# Autodesk Inventor assembly: enc-BackPanel Unten HF-Durchlass - Assembly
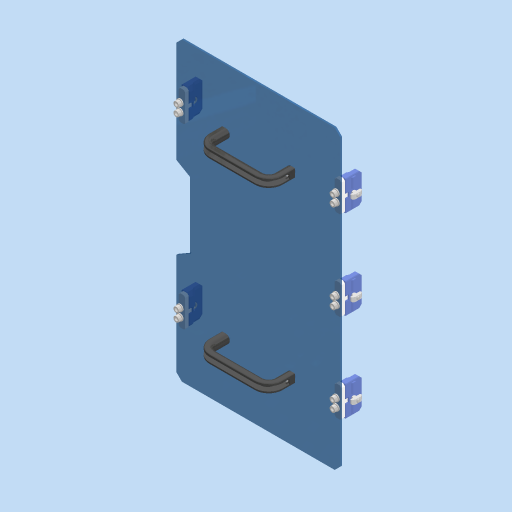
[picture p0: Inventor's stored thumbnail of the model, 512x512]
Saved by Autodesk Inventor 2023.2 (Build 272271000, 271)
## iProperties
Created: 2023-12-04
Part Number: enc-BackPanel Unten HF-Durchlass - Assembly
Document SubType Name: Assembly
Designer: Nils Bade
Author: Nils Bade
## Documents named in this file (4)
- C:\Users\nilsb\Documents\Inventor\Projektarbeit-Bade\Enclosure\enc-BackPanel Unten HF-Durchlass - Assembly.iam
- C:\Users\nilsb\Documents\Inventor\Projektarbeit-Bade\Enclosure\Magnet PanelFrame 90deg connected.iam
- C:\Users\nilsb\Documents\Inventor\Projektarbeit-Bade\Enclosure\item_Handgriff_PA120_Assembly.iam
- C:\Users\nilsb\Documents\Inventor\Projektarbeit-Bade\Enclosure\enc-BackPanel Unten HF-Durchlass.ipt
## Components (8 placed, 3 different names)
1. Magnet PanelFrame 90deg connected:1 [sub-assembly]
2. Magnet PanelFrame 90deg connected:2 [sub-assembly]
3. Magnet PanelFrame 90deg connected:3 [sub-assembly]
4. Magnet PanelFrame 90deg connected:4 [sub-assembly]
5. Magnet PanelFrame 90deg connected:6 [sub-assembly]
6. item_Handgriff_120er:2 [sub-assembly]
7. item_Handgriff_120er:1 [sub-assembly]
8. enc-BackPanel Unten HF-Durchlass:1
## Relationships (21: Mate 21)
- [Mate]: Magnet PanelFrame 90deg connected:4 ↔ enc-BackPanel Unten HF-Durchlass:1
- [Mate]: Magnet PanelFrame 90deg connected:4 ↔ enc-BackPanel Unten HF-Durchlass:1
- [Mate]: Magnet PanelFrame 90deg connected:4 ↔ enc-BackPanel Unten HF-Durchlass:1
- [Mate]: Magnet PanelFrame 90deg connected:6 ↔ enc-BackPanel Unten HF-Durchlass:1
- [Mate]: Magnet PanelFrame 90deg connected:6 ↔ enc-BackPanel Unten HF-Durchlass:1
- [Mate]: Magnet PanelFrame 90deg connected:6 ↔ enc-BackPanel Unten HF-Durchlass:1
- [Mate]: Magnet PanelFrame 90deg connected:1 ↔ enc-BackPanel Unten HF-Durchlass:1
- [Mate]: Magnet PanelFrame 90deg connected:1 ↔ enc-BackPanel Unten HF-Durchlass:1
- [Mate]: Magnet PanelFrame 90deg connected:1 ↔ enc-BackPanel Unten HF-Durchlass:1
- [Mate]: Magnet PanelFrame 90deg connected:2 ↔ enc-BackPanel Unten HF-Durchlass:1
- [Mate]: Magnet PanelFrame 90deg connected:2 ↔ enc-BackPanel Unten HF-Durchlass:1
- [Mate]: Magnet PanelFrame 90deg connected:2 ↔ enc-BackPanel Unten HF-Durchlass:1
- [Mate]: Magnet PanelFrame 90deg connected:3 ↔ enc-BackPanel Unten HF-Durchlass:1
- [Mate]: Magnet PanelFrame 90deg connected:3 ↔ enc-BackPanel Unten HF-Durchlass:1
- [Mate]: Magnet PanelFrame 90deg connected:3 ↔ enc-BackPanel Unten HF-Durchlass:1
- [Mate]: item_Handgriff_120er:2 ↔ enc-BackPanel Unten HF-Durchlass:1
- [Mate]: item_Handgriff_120er:1 ↔ enc-BackPanel Unten HF-Durchlass:1
- [Mate]: item_Handgriff_120er:2 ↔ enc-BackPanel Unten HF-Durchlass:1
- [Mate]: item_Handgriff_120er:1 ↔ enc-BackPanel Unten HF-Durchlass:1
- [Mate]: item_Handgriff_120er:1 ↔ enc-BackPanel Unten HF-Durchlass:1
- [Mate]: item_Handgriff_120er:2 ↔ enc-BackPanel Unten HF-Durchlass:1
